# Autodesk Inventor assembly: Assembly1
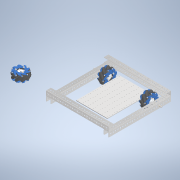
[picture p0: Inventor's stored thumbnail of the model, 180x180]
Saved by Autodesk Inventor 2020 (Build 240168000, 168)
## iProperties
Created: 2019-09-11
Part Number: Assembly1
Document SubType Name: Assembly
Designer: tbloo
Author: tbloo
## Documents named in this file (5)
- D:\Documents\GitHub\AO_Robotics\CAD\Projects\Timothy Bloot\Assembly1.iam
- D:\Documents\GitHub\AO_Robotics\CAD\Parts Kits\FTC Tetrix KOP Organized (7-24-19)\Frame Hardware\Tetrix_39069.ipt
- D:\Documents\GitHub\AO_Robotics\CAD\Parts Kits\FTC Tetrix KOP Organized (7-24-19)\Wheel\Mechanum Wheel\left_a_mecanum wheel.ipt
- D:\Documents\GitHub\AO_Robotics\CAD\Projects\Timothy Bloot\mech_wheel_assembly.iam
- D:\Documents\GitHub\AO_Robotics\CAD\Parts Kits\Created Models\Base Plate.ipt
## Components (8 placed, 4 different names)
1. Tetrix_39069:1 — Rigid:3, Rotational:1
2. Tetrix_39069:2 — Rigid:2
3. Tetrix_39069:3 — Rigid:1, Rigid:3
4. Tetrix_39069:4 — Rigid:1, Rigid:2, Rotational:3
5. left_a_mecanum wheel:2
6. mech_wheel_assembly:1 [sub-assembly] — Rotational:1
7. mech_wheel_assembly:2 [sub-assembly] — Rotational:3
8. Base Plate:1
## Relationships (5: WeldJoint 3, RevoluteJoint 2)
- Rigid:1 [WeldJoint]: Tetrix_39069:3 ↔ Tetrix_39069:4
- Rigid:2 [WeldJoint]: Tetrix_39069:2 ↔ Tetrix_39069:4
- Rigid:3 [WeldJoint]: Tetrix_39069:1 ↔ Tetrix_39069:3
- Rotational:1 [RevoluteJoint]: Tetrix_39069:1 ↔ mech_wheel_assembly:1
- Rotational:3 [RevoluteJoint]: Tetrix_39069:4 ↔ mech_wheel_assembly:2
